# Autodesk Inventor assembly: PIP-Boy 6400 Mk_I Full Assembly
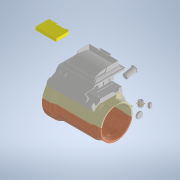
[picture p0: Inventor's stored thumbnail of the model, 180x180]
Saved by Autodesk Inventor 2021 (Build 250183000, 183)
## iProperties
Created: 2021-04-29
Part Number: PIP-Boy 6400 Mk_I Full Assembly
Document SubType Name: Assembly
Designer: trent
Author: trent
## Documents named in this file (5)
- C:\Users\EmeraldLeeTiger\OneDrive - wmpenn.edu\Personal\PIP-Boy 6400 Mk.I\PIP-Boy 6400 Mk_I Full Assembly.iam
- C:\Users\EmeraldLeeTiger\OneDrive - wmpenn.edu\Personal\PIP-Boy 6400 Mk.I\ArmPiece_TopHalf.ipt
- C:\Users\EmeraldLeeTiger\OneDrive - wmpenn.edu\Personal\PIP-Boy 6400 Mk.I\ArmPiece_Lower.ipt
- C:\Users\EmeraldLeeTiger\OneDrive - wmpenn.edu\Personal\PIP-Boy 6400 Mk.I\PIP_Main Unit Subassembly.iam
- C:\Users\EmeraldLeeTiger\OneDrive - wmpenn.edu\Personal\PIP-Boy 6400 Mk.I\Holotape.iam
## Components (4 placed, 4 different names)
1. ArmPiece_TopHalf:1 — Mate:16, Mate:17, Mate:18, Mate:19, Mate:20
2. ArmPiece_Lower:1 — Mate:16, Mate:17
3. PIP_Main Unit Subassembly:1 [sub-assembly] — Mate:18, Mate:19, Mate:20
4. Holotape:1 [sub-assembly]
## Relationships (5: Mate 5)
- Mate:16: ArmPiece_TopHalf:1 ↔ ArmPiece_Lower:1
- Mate:17: ArmPiece_TopHalf:1 ↔ ArmPiece_Lower:1
- Mate:18: ArmPiece_TopHalf:1 ↔ PIP_Main Unit Subassembly:1
- Mate:19: ArmPiece_TopHalf:1 ↔ PIP_Main Unit Subassembly:1
- Mate:20: ArmPiece_TopHalf:1 ↔ PIP_Main Unit Subassembly:1
